# Autodesk Inventor assembly: TopLayerAssembly
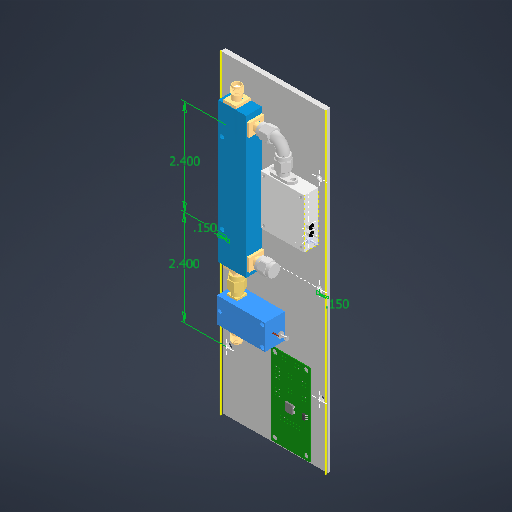
[picture p0: Inventor's stored thumbnail of the model, 512x512]
Saved by Autodesk Inventor 2026.2 (Build 302298010, 298A)
## iProperties
Created: 2026-07-14
Part Number: TopLayerAssembly
Document SubType Name: Assembly
Designer: sonata
Author: sonata
## Documents named in this file (7)
- Z:\crush\mechanical\PAM-modules-mount\TopLayerAssembly.iam
- Z:\crush\mechanical\PAM-modules-mount\BiasTee.iam
- Z:\crush\mechanical\PAM-modules-mount\Coupler.iam
- Z:\crush\mechanical\PAM-modules-mount\PowerDetector.iam
- Z:\crush\mechanical\PAM-modules-mount\PE91492_3D\PE91492_3D\PE91492_3D.ipt
- Z:\crush\mechanical\PAM-modules-mount\PAM_Interface\PAM_Interface\PAM_Interface.ipt
- Z:\crush\mechanical\PAM-modules-mount\TopLayerPlate.ipt
## Components (6 placed, 6 different names)
1. BiasTee:1 [sub-assembly] — Mate:4, Mate:5
2. Coupler:1 [sub-assembly] — Mate:1, Mate:3, Flush:1, Mate:4, Mate:5, Mate:6, Flush:2
3. PowerDetector:1 [sub-assembly] — Mate:2, Mate:3, Flush:1
4. PE91492_3D:1 — Mate:1, Mate:2
5. PAM_Interface:1 — Flush:3
6. TopLayerPlate:1 — Mate:6, Flush:2, Flush:3
## Relationships (9: Mate 6, Flush 3)
- Mate:1: Coupler:1 ↔ PE91492_3D:1
- Mate:2: PowerDetector:1 ↔ PE91492_3D:1
- Mate:3 (8.08 mm): Coupler:1 ↔ PowerDetector:1
- Flush:1 (26.8 mm): Coupler:1 ↔ PowerDetector:1
- Mate:4: BiasTee:1 ↔ Coupler:1
- Mate:5 (17.42 mm): BiasTee:1 ↔ Coupler:1
- Mate:6: Coupler:1 ↔ TopLayerPlate:1
- Flush:2 (-17.78 mm): Coupler:1 ↔ TopLayerPlate:1
- Flush:3 (3.175 mm): PAM_Interface:1 ↔ TopLayerPlate:1
